# Autodesk Inventor assembly: cover완44
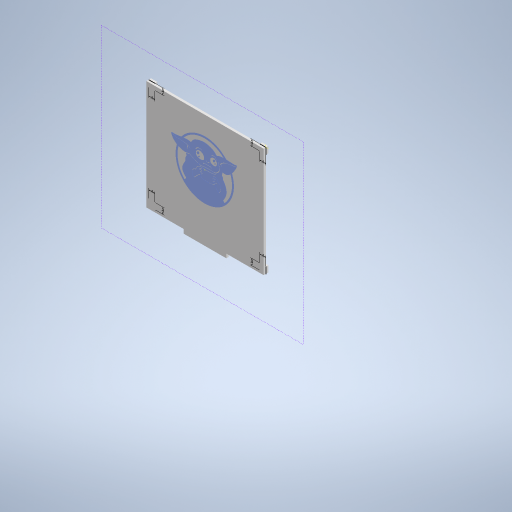
[picture p0: Inventor's stored thumbnail of the model, 512x512]
Saved by Autodesk Inventor 2024 (Build 280153000, 153)
## iProperties
Created: 2024-09-10
Part Number: cover완44
Document SubType Name: Assembly
Designer: pc
Author: pc
## Documents named in this file (3)
- C:\Users\pc\Downloads\cover완44.iam
- C:\Users\pc\Downloads\cover.ipt
- C:\Users\pc\Downloads\YodaDW.ipt
## Components (2 placed, 2 different names)
1. cover:1 — 메이트:1
2. YodaDW:1 — 메이트:1
## Relationships (1: Mate 1)
- 메이트:1 [Mate]: cover:1 ↔ YodaDW:1
